# Autodesk Inventor assembly: capsule.top.assembly
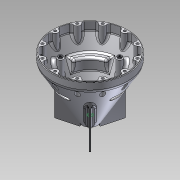
[picture p0: Inventor's stored thumbnail of the model, 180x180]
Saved by Autodesk Inventor 2011 (Build 150239000, 239)
## iProperties
Created: 2011-01-27
Part Number: capsule.top.assembly
Document SubType Name: Assembly
Designer: Casey
Author: Casey
## Documents named in this file (5)
- C:\Users\M. Woods III\Desktop\design\Mechanical Drawings\capsule_top.iam
- C:\Users\M. Woods III\Desktop\design\Mechanical Drawings\capsule_top.ipt
- C:\Users\M. Woods III\Desktop\design\Mechanical Drawings\capsule_fin.ipt
- C:\Users\M. Woods III\Desktop\design\Mechanical Drawings\ANSI B18.3.1M(6)\ANSI B18.3.1M - M3x0.5 x 12(1).ipt
- C:\Users\M. Woods III\Desktop\design\Mechanical Drawings\capsule_contactring.ipt
## Components (11 placed, 4 different names)
1. capsule_top:1 — Tangent:2, Insert:11, Mate:1, Mate:2, Mate:3, Tangent:3, Tangent:4, Mate:4, Mate:5, Mate:6
2. capsule_fin:1 — Tangent:2, Mate:1, Mate:4
3. capsule_fin:2 — Mate:3, Tangent:3, Mate:6
4. capsule_fin:3 — Mate:2, Tangent:4, Mate:5
5. Forged Socket Head Cap Screw - Metric M3x0.5 x 12:1
6. Forged Socket Head Cap Screw - Metric M3x0.5 x 12:2
7. Forged Socket Head Cap Screw - Metric M3x0.5 x 12:3
8. Forged Socket Head Cap Screw - Metric M3x0.5 x 12:4
9. Forged Socket Head Cap Screw - Metric M3x0.5 x 12:5
10. Forged Socket Head Cap Screw - Metric M3x0.5 x 12:6
11. capsule_contactring:1 — Insert:11
## Relationships (10: Mate 6, Tangent 3, Insert 1)
- Tangent:2: capsule_top:1 ↔ capsule_fin:1
- Insert:11: capsule_top:1 ↔ capsule_contactring:1
- Mate:1: capsule_top:1 ↔ capsule_fin:1
- Mate:2: capsule_top:1 ↔ capsule_fin:3
- Mate:3: capsule_top:1 ↔ capsule_fin:2
- Tangent:3: capsule_top:1 ↔ capsule_fin:2
- Tangent:4: capsule_top:1 ↔ capsule_fin:3
- Mate:4: capsule_top:1 ↔ capsule_fin:1
- Mate:5: capsule_top:1 ↔ capsule_fin:3
- Mate:6: capsule_top:1 ↔ capsule_fin:2
